# Autodesk Inventor assembly: Wheel
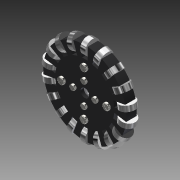
[picture p0: Inventor's stored thumbnail of the model, 180x180]
Saved by Autodesk Inventor 2015 (Build 190159000, 159)
## iProperties
Created: 2016-10-18
Part Number: Wheel
Document SubType Name: Assembly
Designer: James Yelland
Author: James Yelland
## Documents named in this file (10)
- C:\Users\James Yelland\git\LJ-STAND\Design\Models\Wheel\Wheel.iam
- C:\Users\James Yelland\git\LJ-STAND\Design\Models\Wheel\Plate 1.ipt
- C:\Users\James Yelland\git\LJ-STAND\Design\Models\Wheel\Plate 2.ipt
- C:\Users\James Yelland\git\LJ-STAND\Design\Models\Wheel\Plate 3.ipt
- C:\Users\James Yelland\git\LJ-STAND\Design\Models\Wheel\Rod.ipt
- C:\Users\James Yelland\git\LJ-STAND\Design\Models\Wheel\Roller.ipt
- C:\Users\James Yelland\git\LJ-STAND\Design\Models\Wheel\Hub.ipt
- C:\Users\James Yelland\git\LJ-STAND\Design\Models\Wheel\8mm M3 Screw.ipt
- C:\Users\James Yelland\git\LJ-STAND\Design\Models\Wheel\M3 Nut.ipt
- C:\Users\James Yelland\git\LJ-STAND\Design\Models\Wheel\5mm 2-56 Screw.ipt
## Components (52 placed, 9 different names)
1. Plate 1:1 — Insert:1, Insert:2, Tangent:1, Insert:3, Insert:4, Tangent:3, Tangent:6, Tangent:7, Tangent:9, Tangent:11, Tangent:13, Tangent:15, Tangent:17, Tangent:20, Tangent:22, Tangent:23, Tangent:26, Tangent:27, Tangent:29, Tangent:31, Tangent:33, Tangent:35, Tangent:37, Mate:24, Mate:28, Insert:7, Insert:8, Insert:9, Insert:10, Insert:15, Insert:16, Insert:17, Insert:18
2. Plate 2:1 — Insert:1, Insert:2, Mate:1, Tangent:2, Mate:3, Tangent:4, Mate:4, Mate:5, Mate:6, Mate:7, Mate:8, Mate:9, Mate:10, Mate:11, Mate:12, Mate:13, Mate:14, Mate:15, Mate:16, Mate:17, Mate:18, Mate:19, Mate:20, Tangent:5, Tangent:8, Tangent:10, Tangent:12, Tangent:14, Tangent:16, Tangent:18, Tangent:19, Tangent:21, Tangent:24, Tangent:25, Tangent:28, Tangent:30, Tangent:32, Tangent:34, Tangent:36, Tangent:38, Mate:22, Mate:26, Mate:42, Mate:43, Mate:44, Mate:45, Mate:46, Mate:47, Mate:48, Mate:49, Mate:50, Mate:51, Mate:52, Mate:53, Mate:54, Insert:5, Insert:6
3. Plate 3:1 — Insert:5, Insert:6, Insert:11, Insert:12, Insert:13, Insert:14
4. Rod:1 — Tangent:3, Tangent:4, Mate:4, Tangent:7, Tangent:8, Mate:21
5. Roller:1 — Mate:23, Mate:24
6. Rod:2 — Mate:6, Tangent:11, Tangent:12, Mate:40
7. Roller:2 — Mate:25, Mate:26
8. Rod:3 — Mate:7, Tangent:13, Tangent:14, Mate:39
9. Roller:3 — Mate:21, Mate:22
10. Rod:4 — Mate:8, Tangent:15, Tangent:16, Mate:38
11. Roller:4 — Mate:29, Mate:42
12. Rod:5 — Mate:14, Tangent:27, Tangent:28, Mate:32
13. Roller:5 — Mate:33, Mate:46
14. Rod:6 — Mate:16, Tangent:31, Tangent:32, Mate:30
15. Roller:6 — Mate:40, Mate:53
16. Rod:7 — Mate:10, Tangent:19, Tangent:20, Mate:36
17. Roller:7 — Mate:34, Mate:47
18. Rod:8 — Mate:5, Tangent:9, Tangent:10, Mate:41
19. Roller:8 — Mate:27, Mate:28
20. Rod:9 — Mate:13, Tangent:25, Tangent:26, Mate:33
21. Roller:9 — Mate:35, Mate:48
22. Rod:10 — Mate:15, Tangent:29, Tangent:30, Mate:31
23. Roller:10 — Mate:41, Mate:54
24. Rod:11 — Mate:17, Tangent:33, Tangent:34, Mate:29
25. Roller:11 — Mate:39, Mate:52
26. Rod:12 — Mate:20, Tangent:5, Tangent:6, Mate:23
27. Roller:12 — Mate:37, Mate:50
28. Rod:13 — Mate:19, Tangent:37, Tangent:38, Mate:25
29. Roller:13 — Mate:36, Mate:49
30. Rod:14 — Mate:18, Tangent:35, Tangent:36, Mate:27
31. Roller:14 — Mate:38, Mate:51
32. Rod:15 — Mate:11, Tangent:21, Tangent:22, Mate:35
33. Roller:15 — Mate:32, Mate:45
34. Rod:16 — Mate:12, Tangent:23, Tangent:24, Mate:34
35. Roller:16 — Mate:31, Mate:44
36. Rod:17 — Mate:9, Tangent:17, Tangent:18, Mate:37
37. Roller:17 — Mate:30, Mate:43
38. Rod:18 — Tangent:1, Mate:1, Tangent:2, Mate:2
39. Roller:18 — Mate:2, Mate:3
40. Hub:1 — Insert:3, Insert:4
41. 8mm M3 Screw:1 — Insert:10
42. 8mm M3 Screw:2 — Insert:9
43. 8mm M3 Screw:3 — Insert:8
44. 8mm M3 Screw:4 — Insert:7
45. M3 Nut:1 — Insert:11
46. M3 Nut:2 — Insert:14
47. M3 Nut:3 — Insert:12
48. M3 Nut:4 — Insert:13
49. 5mm 2-56 Screw:1 — Insert:15
50. 5mm 2-56 Screw:2 — Insert:18
51. 5mm 2-56 Screw:3 — Insert:17
52. 5mm 2-56 Screw:4 — Insert:16
## Relationships (110: Mate 54, Tangent 38, Insert 18)
- Insert:1: Plate 1:1 ↔ Plate 2:1
- Insert:2: Plate 1:1 ↔ Plate 2:1
- Tangent:1: Plate 1:1 ↔ Rod:18
- Mate:1: Plate 2:1 ↔ Rod:18
- Tangent:2: Plate 2:1 ↔ Rod:18
- Mate:2: Rod:18 ↔ Roller:18
- Mate:3 (0.1 mm): Plate 2:1 ↔ Roller:18
- Insert:3: Plate 1:1 ↔ Hub:1
- Insert:4: Plate 1:1 ↔ Hub:1
- Tangent:3: Plate 1:1 ↔ Rod:1
- Tangent:4: Plate 2:1 ↔ Rod:1
- Mate:4: Plate 2:1 ↔ Rod:1
- Mate:5: Plate 2:1 ↔ Rod:8
- Mate:6: Plate 2:1 ↔ Rod:2
- Mate:7: Plate 2:1 ↔ Rod:3
- Mate:8: Plate 2:1 ↔ Rod:4
- Mate:9: Plate 2:1 ↔ Rod:17
- Mate:10: Plate 2:1 ↔ Rod:7
- Mate:11: Plate 2:1 ↔ Rod:15
- Mate:12: Plate 2:1 ↔ Rod:16
- Mate:13: Plate 2:1 ↔ Rod:9
- Mate:14: Plate 2:1 ↔ Rod:5
- Mate:15: Plate 2:1 ↔ Rod:10
- Mate:16: Plate 2:1 ↔ Rod:6
- Mate:17: Plate 2:1 ↔ Rod:11
- Mate:18: Plate 2:1 ↔ Rod:14
- Mate:19: Plate 2:1 ↔ Rod:13
- Mate:20: Plate 2:1 ↔ Rod:12
- Tangent:5: Plate 2:1 ↔ Rod:12
- Tangent:6: Plate 1:1 ↔ Rod:12
- Tangent:7: Plate 1:1 ↔ Rod:1
- Tangent:8: Plate 2:1 ↔ Rod:1
- Tangent:9: Plate 1:1 ↔ Rod:8
- Tangent:10: Plate 2:1 ↔ Rod:8
- Tangent:11: Plate 1:1 ↔ Rod:2
- Tangent:12: Plate 2:1 ↔ Rod:2
- Tangent:13: Plate 1:1 ↔ Rod:3
- Tangent:14: Plate 2:1 ↔ Rod:3
- Tangent:15: Plate 1:1 ↔ Rod:4
- Tangent:16: Plate 2:1 ↔ Rod:4
- Tangent:17: Plate 1:1 ↔ Rod:17
- Tangent:18: Plate 2:1 ↔ Rod:17
- Tangent:19: Plate 2:1 ↔ Rod:7
- Tangent:20: Plate 1:1 ↔ Rod:7
- Tangent:21: Plate 2:1 ↔ Rod:15
- Tangent:22: Plate 1:1 ↔ Rod:15
- Tangent:23: Plate 1:1 ↔ Rod:16
- Tangent:24: Plate 2:1 ↔ Rod:16
- Tangent:25: Plate 2:1 ↔ Rod:9
- Tangent:26: Plate 1:1 ↔ Rod:9
- Tangent:27: Plate 1:1 ↔ Rod:5
- Tangent:28: Plate 2:1 ↔ Rod:5
- Tangent:29: Plate 1:1 ↔ Rod:10
- Tangent:30: Plate 2:1 ↔ Rod:10
- Tangent:31: Plate 1:1 ↔ Rod:6
- Tangent:32: Plate 2:1 ↔ Rod:6
- Tangent:33: Plate 1:1 ↔ Rod:11
- Tangent:34: Plate 2:1 ↔ Rod:11
- Tangent:35: Plate 1:1 ↔ Rod:14
- Tangent:36: Plate 2:1 ↔ Rod:14
- Tangent:37: Plate 1:1 ↔ Rod:13
- Tangent:38: Plate 2:1 ↔ Rod:13
- Mate:21: Rod:1 ↔ Roller:3
- Mate:22 (0.1 mm): Plate 2:1 ↔ Roller:3
- Mate:23: Roller:1 ↔ Rod:12
- Mate:24 (0.1 mm): Plate 1:1 ↔ Roller:1
- Mate:25: Roller:2 ↔ Rod:13
- Mate:26 (0.1 mm): Plate 2:1 ↔ Roller:2
- Mate:27: Roller:8 ↔ Rod:14
- Mate:28 (0.1 mm): Plate 1:1 ↔ Roller:8
- Mate:29: Roller:4 ↔ Rod:11
- Mate:30: Rod:6 ↔ Roller:17
- Mate:31: Rod:10 ↔ Roller:16
- Mate:32: Rod:5 ↔ Roller:15
- Mate:33: Roller:5 ↔ Rod:9
- Mate:34: Roller:7 ↔ Rod:16
- Mate:35: Roller:9 ↔ Rod:15
- Mate:36: Rod:7 ↔ Roller:13
- Mate:37: Roller:12 ↔ Rod:17
- Mate:38: Rod:4 ↔ Roller:14
- Mate:39: Rod:3 ↔ Roller:11
- Mate:40: Rod:2 ↔ Roller:6
- Mate:41: Rod:8 ↔ Roller:10
- Mate:42 (0.1 mm): Plate 2:1 ↔ Roller:4
- Mate:43 (0.1 mm): Plate 2:1 ↔ Roller:17
- Mate:44 (0.1 mm): Plate 2:1 ↔ Roller:16
- Mate:45 (0.1 mm): Plate 2:1 ↔ Roller:15
- Mate:46 (0.1 mm): Plate 2:1 ↔ Roller:5
- Mate:47 (0.1 mm): Plate 2:1 ↔ Roller:7
- Mate:48 (0.1 mm): Plate 2:1 ↔ Roller:9
- Mate:49 (0.1 mm): Plate 2:1 ↔ Roller:13
- Mate:50 (0.1 mm): Plate 2:1 ↔ Roller:12
- Mate:51 (0.1 mm): Plate 2:1 ↔ Roller:14
- Mate:52 (0.1 mm): Plate 2:1 ↔ Roller:11
- Mate:53 (0.1 mm): Plate 2:1 ↔ Roller:6
- Mate:54 (0.1 mm): Plate 2:1 ↔ Roller:10
- Insert:5: Plate 2:1 ↔ Plate 3:1
- Insert:6: Plate 2:1 ↔ Plate 3:1
- Insert:7: Plate 1:1 ↔ 8mm M3 Screw:4
- Insert:8: Plate 1:1 ↔ 8mm M3 Screw:3
- Insert:9: Plate 1:1 ↔ 8mm M3 Screw:2
- Insert:10: Plate 1:1 ↔ 8mm M3 Screw:1
- Insert:11: Plate 3:1 ↔ M3 Nut:1
- Insert:12: Plate 3:1 ↔ M3 Nut:3
- Insert:13: Plate 3:1 ↔ M3 Nut:4
- Insert:14: Plate 3:1 ↔ M3 Nut:2
- Insert:15: Plate 1:1 ↔ 5mm 2-56 Screw:1
- Insert:16: Plate 1:1 ↔ 5mm 2-56 Screw:4
- Insert:17: Plate 1:1 ↔ 5mm 2-56 Screw:3
- Insert:18: Plate 1:1 ↔ 5mm 2-56 Screw:2
